# Autodesk Inventor assembly: ESC_Assembly
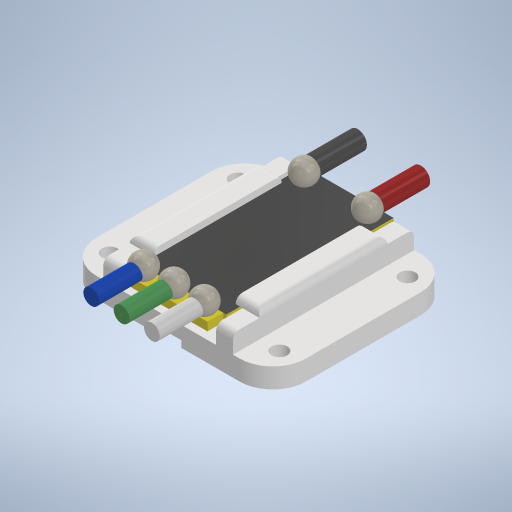
[picture p0: Inventor's stored thumbnail of the model, 512x512]
Saved by Autodesk Inventor 2024 (Build 280153000, 153)
## iProperties
Created: 2023-04-14
Part Number: ESC_Assembly
Document SubType Name: Assembly
Designer: richb366163
Author: richb366163
## Documents named in this file (3)
- C:\Users\18179\Desktop\TuppyMkIV\ESC_Assembly.iam
- C:\Users\18179\Desktop\TuppyMkIV\BESC30-R3.ipt
- C:\Users\18179\Desktop\TuppyMkIV\ESC_Mount.ipt
## Components (2 placed, 2 different names)
1. BESC30-R3:1 — Mate:1
2. ESC_Mount:1 — Mate:1
## Relationships (1: Mate 1)
- Mate:1: BESC30-R3:1 ↔ ESC_Mount:1
